# Autodesk Inventor assembly: 总装配
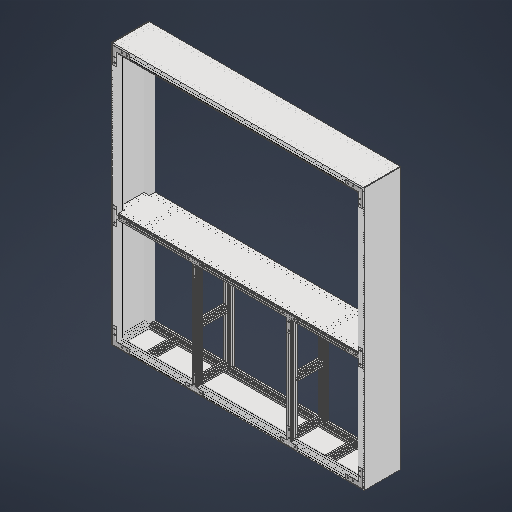
[picture p0: Inventor's stored thumbnail of the model, 512x512]
Saved by Autodesk Inventor 2025 (Build 290162000, 162)
## iProperties
Created: 2025-06-18
Part Number: 总装配
Document SubType Name: Assembly
Designer: XH
Author: XH
## Documents named in this file (13)
- D:\2 B Mechanical design\Volkswagen_ID\总装配.iam
- D:\2 B Mechanical design\Volkswagen_ID\后座大小\零件1.ipt
- D:\2 B Mechanical design\Volkswagen_ID\2020铝型材\框架.ipt
- D:\2 B Mechanical design\Volkswagen_ID\2020铝型材\铝方管2020x.ipt
- D:\2 B Mechanical design\Volkswagen_ID\CAD\板材加工step\板材.ipt
- D:\2 B Mechanical design\Volkswagen_ID\CAD\板材加工step\板材2.ipt
- D:\2 B Mechanical design\Volkswagen_ID\2020铝型材\铝方管2020x60.ipt
- D:\2 B Mechanical design\Volkswagen_ID\CAD\板材加工step\内板.ipt
- D:\2 B Mechanical design\Volkswagen_ID\CAD\板材加工step\板材后.ipt
- D:\2 B Mechanical design\Volkswagen_ID\2020铝型材\铝方管2020中.ipt
- D:\2 B Mechanical design\Volkswagen_ID\2020铝型材\铝方管2020x2.ipt
- D:\2 B Mechanical design\Volkswagen_ID\转接件\T型.ipt
- D:\2 B Mechanical design\Volkswagen_ID\转接件\L型.ipt
## Components (48 placed, 12 different names)
1. 零件1:1 — 表面齐平:14
2. 铝方管2020中:1 — 配合:33, 表面齐平:33, 表面齐平:34, 配合:39, 表面齐平:41, 表面齐平:42, 配合:47, 配合:48, 配合:50, 配合:51, 相切:1, 相切:2, 相切:3, 相切:4, 相切:7, 配合:53, 相切:12, 配合:74, 配合:75
3. 铝方管2020中:2 — 表面齐平:34, 配合:34, 表面齐平:35, 表面齐平:38, 表面齐平:46, 表面齐平:52, 配合:64, 配合:68, 表面齐平:69, 表面齐平:70
4. 铝方管2020x60:6 — 配合:36, 表面齐平:37, 表面齐平:38
5. 铝方管2020x2:1 — 表面齐平:42, 表面齐平:43, 配合:50, 配合:52, 相切:8, 配合:54, 相切:15, 表面齐平:53, 表面齐平:56, 配合:62, 表面齐平:59, 配合:65, 表面齐平:65, 配合:71
6. 铝方管2020x2:2 — 表面齐平:43, 配合:51, 相切:9, 相切:16, 表面齐平:54, 表面齐平:62, 配合:72, 表面齐平:66
7. 铝方管2020x60:8 — 配合:43, 表面齐平:46, 表面齐平:47
8. T型:1 — 配合:46, 相切:5, 相切:6, 相切:7
9. T型:2 — 配合:47, 相切:1, 相切:2, 相切:8
10. T型:3 — 配合:48, 相切:3, 相切:4, 相切:9
11. T型:4 — 配合:53, 相切:10, 相切:11, 相切:12
12. T型:5 — 配合:54, 相切:13, 相切:14, 相切:15
13. T型:6 — 配合:55, 相切:16, 相切:17, 相切:18
14. L型:1 — 配合:56, 相切:19, 相切:20, 相切:21
15. L型:2 — 配合:58
16. L型:3 — 配合:59
17. L型:4 — 配合:57
18. 铝方管2020x2:3 — 配合:60, 表面齐平:52, 表面齐平:53, 表面齐平:58
19. 铝方管2020x2:4 — 表面齐平:54, 配合:61, 表面齐平:55, 表面齐平:60, 表面齐平:61, 配合:66, 配合:67
20. 铝方管2020x60:11 — 表面齐平:56, 配合:62, 表面齐平:58
21. 铝方管2020x60:12 — 配合:63, 表面齐平:57, 表面齐平:71
22. 铝方管2020x60:13 — 配合:64, 表面齐平:59, 配合:65
23. 铝方管2020x60:14 — 表面齐平:60, 表面齐平:61, 配合:66
24. 铝方管2020x60:15 — 配合:67, 配合:68, 表面齐平:62
25. 铝方管2020x:5 — 表面齐平:63, 配合:69, 表面齐平:64, 配合:70
26. 铝方管2020x60:16 — 表面齐平:65, 配合:71, 表面齐平:67
27. 铝方管2020x60:17 — 配合:72, 表面齐平:66, 表面齐平:67
28. 铝方管2020x60:18 — 表面齐平:68, 配合:73, 表面齐平:72
29. 铝方管2020x60:19 — 配合:74, 表面齐平:69, 表面齐平:72
30. 铝方管2020x60:20 — 表面齐平:70, 配合:75, 表面齐平:71
31. 板材后:1 — 配合:31, 配合:32, 表面齐平:32
32. 内板:1 — 配合:28, 表面齐平:30
33. 板材:1 — 配合:6, 表面齐平:15, 表面齐平:17, 配合:9, 表面齐平:18, 表面齐平:19, 配合:17, 配合:20, 表面齐平:32
34. 板材:2 — 配合:7, 表面齐平:16, 表面齐平:17, 表面齐平:20, 配合:15, 配合:23, 配合:26, 配合:32
35. 内板:3 — 配合:39, 表面齐平:41
36. 板材2:1 — 配合:8, 配合:9, 表面齐平:18, 表面齐平:19, 表面齐平:20, 配合:14, 配合:16, 配合:25, 表面齐平:29
37. 框架:1 — 表面齐平:4, 表面齐平:5, 表面齐平:7, 表面齐平:10, 配合:4, 配合:5, 表面齐平:12, 表面齐平:13, 配合:6, 表面齐平:15, 配合:43, 表面齐平:47
38. 框架:2 — 表面齐平:4, 表面齐平:5, 表面齐平:11, 配合:7, 表面齐平:16, 表面齐平:35, 表面齐平:37, 配合:70
39. 铝方管2020x:1 — 表面齐平:7, 表面齐平:10, 配合:4, 表面齐平:11, 配合:60, 配合:61, 表面齐平:55
40. 铝方管2020x:2 — 配合:5, 表面齐平:12, 表面齐平:13, 表面齐平:14, 配合:8
41. 铝方管2020x:3 — 配合:21, 配合:24, 配合:31, 配合:52, 相切:13, 相切:14, 配合:55, 相切:17, 相切:18, 配合:58, 配合:59, 配合:63, 表面齐平:57, 表面齐平:63, 表面齐平:68, 配合:73
42. 铝方管2020x:4 — 配合:14, 配合:18, 配合:27, 表面齐平:29, 配合:28, 表面齐平:30, 配合:56, 相切:19, 配合:57
43. 框架:3 — 相切:10, 相切:11, 相切:20, 相切:21
44. 框架:4 — 配合:15, 配合:33, 表面齐平:33, 配合:34, 配合:36, 配合:46, 相切:5, 相切:6
45. 铝方管2020x60:1 — 配合:16, 配合:17, 配合:18
46. 铝方管2020x60:2 — 配合:20, 配合:21
47. 铝方管2020x60:3 — 配合:23, 配合:24, 配合:69, 表面齐平:64
48. 铝方管2020x60:4 — 配合:25, 配合:26, 配合:27
## Relationships (133: Mate 57, Flush 55, Tangent 21)
- 表面齐平:4 [Flush]: 框架:1 ↔ 框架:2
- 表面齐平:5 [Flush]: 框架:1 ↔ 框架:2
- 表面齐平:7 [Flush]: 框架:1 ↔ 铝方管2020x:1
- 表面齐平:10 [Flush]: 框架:1 ↔ 铝方管2020x:1
- 配合:4 [Mate]: 框架:1 ↔ 铝方管2020x:1
- 表面齐平:11 [Flush]: 框架:2 ↔ 铝方管2020x:1
- 配合:5 [Mate]: 框架:1 ↔ 铝方管2020x:2
- 表面齐平:12 [Flush]: 框架:1 ↔ 铝方管2020x:2
- 表面齐平:13 [Flush]: 框架:1 ↔ 铝方管2020x:2
- 表面齐平:14 [Flush]: 零件1:1 ↔ 铝方管2020x:2
- 配合:6 [Mate]: 板材:1 ↔ 框架:1
- 表面齐平:15 [Flush]: 板材:1 ↔ 框架:1
- 配合:7 [Mate]: 板材:2 ↔ 框架:2
- 表面齐平:16 [Flush]: 板材:2 ↔ 框架:2
- 表面齐平:17 [Flush]: 板材:1 ↔ 板材:2
- 配合:8 [Mate]: 板材2:1 ↔ 铝方管2020x:2
- 配合:9 [Mate]: 板材:1 ↔ 板材2:1
- 表面齐平:18 [Flush]: 板材:1 ↔ 板材2:1
- 表面齐平:19 [Flush]: 板材:1 ↔ 板材2:1
- 表面齐平:20 [Flush]: 板材:2 ↔ 板材2:1
- [Flush]: 框架:3 ↔ 框架:4
- [Flush]: 框架:3 ↔ 框架:4
- [Flush]: 铝方管2020x:3 ↔ 框架:3
- [Flush]: 铝方管2020x:3 ↔ 框架:3
- [Mate]: 铝方管2020x:3 ↔ 框架:3
- [Flush]: 铝方管2020x:3 ↔ 框架:4
- [Mate]: 铝方管2020x:4 ↔ 框架:3
- [Flush]: 铝方管2020x:4 ↔ 框架:3
- [Flush]: 铝方管2020x:4 ↔ 框架:3
- 配合:14 [Mate]: 板材2:1 ↔ 铝方管2020x:4
- 配合:15 [Mate]: 板材:2 ↔ 框架:4
- 配合:16 [Mate]: 板材2:1 ↔ 铝方管2020x60:1
- 配合:17 [Mate]: 板材:1 ↔ 铝方管2020x60:1
- 配合:18 [Mate]: 铝方管2020x:4 ↔ 铝方管2020x60:1
- 配合:20 [Mate]: 板材:1 ↔ 铝方管2020x60:2
- 配合:21 [Mate]: 铝方管2020x:3 ↔ 铝方管2020x60:2
- 配合:23 [Mate]: 板材:2 ↔ 铝方管2020x60:3
- 配合:24 [Mate]: 铝方管2020x:3 ↔ 铝方管2020x60:3
- 配合:25 [Mate]: 板材2:1 ↔ 铝方管2020x60:4
- 配合:26 [Mate]: 板材:2 ↔ 铝方管2020x60:4
- 配合:27 [Mate]: 铝方管2020x:4 ↔ 铝方管2020x60:4
- 表面齐平:29 [Flush]: 板材2:1 ↔ 铝方管2020x:4
- 配合:28 [Mate]: 内板:1 ↔ 铝方管2020x:4
- 表面齐平:30 [Flush]: 内板:1 ↔ 铝方管2020x:4
- 配合:31 [Mate]: 板材后:1 ↔ 铝方管2020x:3
- 配合:32 [Mate]: 板材后:1 ↔ 板材:2
- 表面齐平:32 [Flush]: 板材后:1 ↔ 板材:1
- 配合:33 [Mate]: 铝方管2020中:1 ↔ 框架:4
- 表面齐平:33 [Flush]: 铝方管2020中:1 ↔ 框架:4
- 表面齐平:34 [Flush]: 铝方管2020中:1 ↔ 铝方管2020中:2
- 配合:34 [Mate]: 铝方管2020中:2 ↔ 框架:4
- 表面齐平:35 [Flush]: 铝方管2020中:2 ↔ 框架:2
- 配合:36 [Mate]: 铝方管2020x60:6 ↔ 框架:4
- 表面齐平:37 [Flush]: 铝方管2020x60:6 ↔ 框架:2
- 表面齐平:38 [Flush]: 铝方管2020中:2 ↔ 铝方管2020x60:6
- 配合:39 [Mate]: 铝方管2020中:1 ↔ 内板:3
- 表面齐平:41 [Flush]: 铝方管2020中:1 ↔ 内板:3
- 表面齐平:42 [Flush]: 铝方管2020中:1 ↔ 铝方管2020x2:1
- 表面齐平:43 [Flush]: 铝方管2020x2:1 ↔ 铝方管2020x2:2
- 配合:43 [Mate]: 铝方管2020x60:8 ↔ 框架:1
- 表面齐平:46 [Flush]: 铝方管2020中:2 ↔ 铝方管2020x60:8
- 表面齐平:47 [Flush]: 铝方管2020x60:8 ↔ 框架:1
- 配合:46 [Mate]: T型:1 ↔ 框架:4
- 配合:47 [Mate]: 铝方管2020中:1 ↔ T型:2
- 配合:48 [Mate]: 铝方管2020中:1 ↔ T型:3
- 配合:50 [Mate]: 铝方管2020中:1 ↔ 铝方管2020x2:1
- 配合:51 [Mate]: 铝方管2020中:1 ↔ 铝方管2020x2:2
- 配合:52 [Mate]: 铝方管2020x2:1 ↔ 铝方管2020x:3
- 相切:1 [Tangent]: 铝方管2020中:1 ↔ T型:2
- 相切:2 [Tangent]: 铝方管2020中:1 ↔ T型:2
- 相切:3 [Tangent]: 铝方管2020中:1 ↔ T型:3
- 相切:4 [Tangent]: 铝方管2020中:1 ↔ T型:3
- 相切:5 [Tangent]: T型:1 ↔ 框架:4
- 相切:6 [Tangent]: T型:1 ↔ 框架:4
- 相切:7 [Tangent]: 铝方管2020中:1 ↔ T型:1
- 相切:8 [Tangent]: 铝方管2020x2:1 ↔ T型:2
- 相切:9 [Tangent]: 铝方管2020x2:2 ↔ T型:3
- 配合:53 [Mate]: 铝方管2020中:1 ↔ T型:4
- 相切:10 [Tangent]: T型:4 ↔ 框架:3
- 相切:11 [Tangent]: T型:4 ↔ 框架:3
- 相切:12 [Tangent]: 铝方管2020中:1 ↔ T型:4
- 配合:54 [Mate]: 铝方管2020x2:1 ↔ T型:5
- 相切:13 [Tangent]: T型:5 ↔ 铝方管2020x:3
- 相切:14 [Tangent]: T型:5 ↔ 铝方管2020x:3
- 相切:15 [Tangent]: 铝方管2020x2:1 ↔ T型:5
- 配合:55 [Mate]: T型:6 ↔ 铝方管2020x:3
- 相切:16 [Tangent]: 铝方管2020x2:2 ↔ T型:6
- 相切:17 [Tangent]: T型:6 ↔ 铝方管2020x:3
- 相切:18 [Tangent]: T型:6 ↔ 铝方管2020x:3
- 配合:56 [Mate]: L型:1 ↔ 铝方管2020x:4
- 相切:19 [Tangent]: L型:1 ↔ 铝方管2020x:4
- 相切:20 [Tangent]: L型:1 ↔ 框架:3
- 相切:21 [Tangent]: L型:1 ↔ 框架:3
- 配合:57 [Mate]: L型:4 ↔ 铝方管2020x:4
- 配合:58 [Mate]: L型:2 ↔ 铝方管2020x:3
- 配合:59 [Mate]: L型:3 ↔ 铝方管2020x:3
- 配合:60 [Mate]: 铝方管2020x2:3 ↔ 铝方管2020x:1
- 表面齐平:52 [Flush]: 铝方管2020中:2 ↔ 铝方管2020x2:3
- 表面齐平:53 [Flush]: 铝方管2020x2:1 ↔ 铝方管2020x2:3
- 表面齐平:54 [Flush]: 铝方管2020x2:2 ↔ 铝方管2020x2:4
- 配合:61 [Mate]: 铝方管2020x2:4 ↔ 铝方管2020x:1
- 表面齐平:55 [Flush]: 铝方管2020x2:4 ↔ 铝方管2020x:1
- 表面齐平:56 [Flush]: 铝方管2020x2:1 ↔ 铝方管2020x60:11
- 配合:62 [Mate]: 铝方管2020x2:1 ↔ 铝方管2020x60:11
- 配合:63 [Mate]: 铝方管2020x60:12 ↔ 铝方管2020x:3
- 表面齐平:57 [Flush]: 铝方管2020x60:12 ↔ 铝方管2020x:3
- 表面齐平:58 [Flush]: 铝方管2020x2:3 ↔ 铝方管2020x60:11
- 配合:64 [Mate]: 铝方管2020中:2 ↔ 铝方管2020x60:13
- 表面齐平:59 [Flush]: 铝方管2020x2:1 ↔ 铝方管2020x60:13
- 配合:65 [Mate]: 铝方管2020x2:1 ↔ 铝方管2020x60:13
- 表面齐平:60 [Flush]: 铝方管2020x2:4 ↔ 铝方管2020x60:14
- 表面齐平:61 [Flush]: 铝方管2020x2:4 ↔ 铝方管2020x60:14
- 配合:66 [Mate]: 铝方管2020x2:4 ↔ 铝方管2020x60:14
- 配合:67 [Mate]: 铝方管2020x2:4 ↔ 铝方管2020x60:15
- 配合:68 [Mate]: 铝方管2020中:2 ↔ 铝方管2020x60:15
- 表面齐平:62 [Flush]: 铝方管2020x2:2 ↔ 铝方管2020x60:15
- 表面齐平:63 [Flush]: 铝方管2020x:5 ↔ 铝方管2020x:3
- 配合:69 [Mate]: 铝方管2020x:5 ↔ 铝方管2020x60:3
- 表面齐平:64 [Flush]: 铝方管2020x:5 ↔ 铝方管2020x60:3
- 配合:70 [Mate]: 铝方管2020x:5 ↔ 框架:2
- 表面齐平:65 [Flush]: 铝方管2020x2:1 ↔ 铝方管2020x60:16
- 配合:71 [Mate]: 铝方管2020x2:1 ↔ 铝方管2020x60:16
- 配合:72 [Mate]: 铝方管2020x2:2 ↔ 铝方管2020x60:17
- 表面齐平:66 [Flush]: 铝方管2020x2:2 ↔ 铝方管2020x60:17
- 表面齐平:67 [Flush]: 铝方管2020x60:16 ↔ 铝方管2020x60:17
- 表面齐平:68 [Flush]: 铝方管2020x60:18 ↔ 铝方管2020x:3
- 配合:73 [Mate]: 铝方管2020x60:18 ↔ 铝方管2020x:3
- 配合:74 [Mate]: 铝方管2020中:1 ↔ 铝方管2020x60:19
- 表面齐平:69 [Flush]: 铝方管2020中:2 ↔ 铝方管2020x60:19
- 表面齐平:70 [Flush]: 铝方管2020中:2 ↔ 铝方管2020x60:20
- 配合:75 [Mate]: 铝方管2020中:1 ↔ 铝方管2020x60:20
- 表面齐平:71 [Flush]: 铝方管2020x60:12 ↔ 铝方管2020x60:20
- 表面齐平:72 [Flush]: 铝方管2020x60:18 ↔ 铝方管2020x60:19
## Named parameters: d33_d3 = 0 mm, d34_d4 = 0 mm, d35_d8 = 0 mm, d36_d12 = 0 mm, d37_d13 = 0 mm, d38_d14 = 0 mm, d39_d15 = 0 mm, d40_d16 = 0 mm, d41_d17 = 0 mm
